# Autodesk Inventor assembly: podwojne koło zebate drugi skręt_MIR
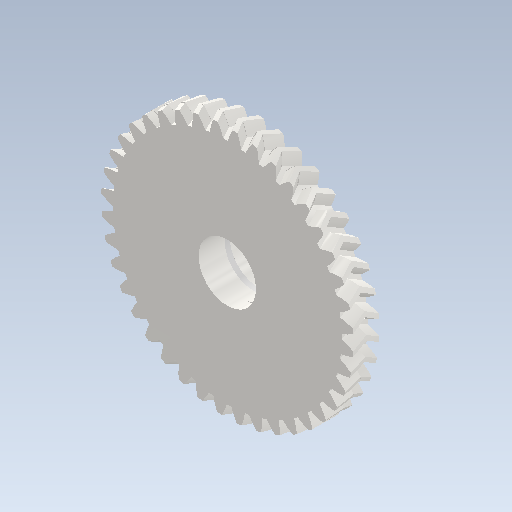
[picture p0: Inventor's stored thumbnail of the model, 512x512]
Saved by Autodesk Inventor 2021 (Build 250183000, 183)
## iProperties
Created: 2021-06-27
Part Number: podwojne koło zebate drugi skręt_MIR
Document SubType Name: Assembly
Designer: Łukasz
Author: Łukasz
## Documents named in this file (4)
- E:\GITHUB_Czołg\Szybki-Czolg-antyRadziecki\koła zębate\Design Accelerator\podwojne koło zebate drugi skręt_MIR.iam
- E:\GITHUB_Czołg\Szybki-Czolg-antyRadziecki\koła zębate\Design Accelerator\inny set zebow\Design Accelerator\Spur Gear11_MIR.ipt
- E:\GITHUB_Czołg\Szybki-Czolg-antyRadziecki\podkładka_MIR.ipt
- E:\GITHUB_Czołg\Szybki-Czolg-antyRadziecki\koła zębate\Design Accelerator\inny set zebow\Design Accelerator\Spur Gear21 bez spacera2_MIR.ipt
## Components (3 placed, 3 different names)
1. Spur Gear11_MIR:1 — Rigid:1
2. podkładka_MIR:1 — Rigid:1, Rotational:1
3. Spur Gear21 bez spacera2_MIR:1 — Rotational:1
## Relationships (2: WeldJoint 1, RevoluteJoint 1)
- Rigid:1 [WeldJoint]: Spur Gear11_MIR:1 ↔ podkładka_MIR:1
- Rotational:1 [RevoluteJoint]: podkładka_MIR:1 ↔ Spur Gear21 bez spacera2_MIR:1
